# Autodesk Inventor assembly: NDV-1000 Center 01
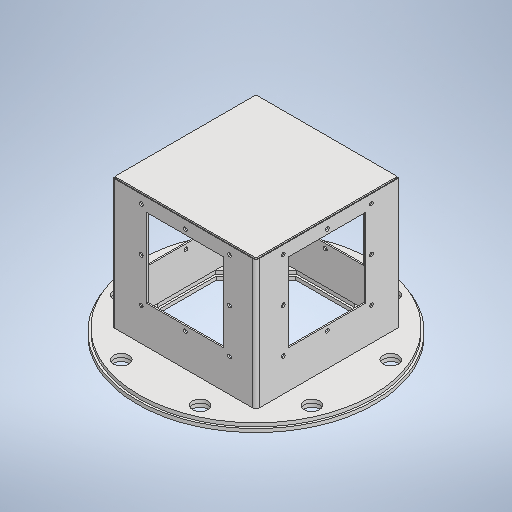
[picture p0: Inventor's stored thumbnail of the model, 512x512]
Saved by Autodesk Inventor 2026.2 (Build 302298000, 298)
## iProperties
Created: 2026-05-12
Part Number: NDV-1000 Center 01
Document SubType Name: Assembly
Designer: admin
Stock Number: Центр
Author: admin
## Documents named in this file (5)
- C:\Users\admin\Documents\Inventor\NDV-DistribSystem\DRS_D1200\NDV-1000 Center 01.iam
- C:\Users\admin\Documents\Inventor\NDV-DistribSystem\DRS_D1200\NDV-1103 Center flange 01.ipt
- C:\Users\admin\Documents\Inventor\NDV-DistribSystem\DRS_D1200\NDV-1101 Center wall 01.ipt
- C:\Users\admin\Documents\Inventor\NDV-DistribSystem\DRS_D1200\NDV-1102 Center cap 01.ipt
- C:\Users\admin\Documents\Inventor\NDV-DistribSystem\DRS_D1200\NDV-1104 Center flange top 01.ipt
## Components (5 placed, 4 different names)
1. NDV-1103 Center flange 01:1 — Mate:6, Flush:3, Flush:4, Flush:5, Flush:6, Mate:9, Mate:10, Flush:7, Flush:8
2. NDV-1101 Center wall 01:1 — Mate:10, Rigid:22, Flush:5, Flush:6, Mate:8
3. NDV-1101 Center wall 01:2 — Rigid:22, Mate:7, Mate:9, Mate:10
4. NDV-1102 Center cap 01:1 — Mate:10, Flush:7, Flush:8
5. NDV-1104 Center flange top 01:1 — Mate:6, Flush:3, Flush:4, Mate:7, Mate:8
## Relationships (13: Mate 6, Flush 6, WeldJoint 1)
- Mate:10: NDV-1101 Center wall 01:1 ↔ NDV-1102 Center cap 01:1
- Rigid:22 [WeldJoint]: NDV-1101 Center wall 01:1 ↔ NDV-1101 Center wall 01:2
- Mate:6: NDV-1103 Center flange 01:1 ↔ NDV-1104 Center flange top 01:1
- Flush:3: NDV-1103 Center flange 01:1 ↔ NDV-1104 Center flange top 01:1
- Flush:4: NDV-1103 Center flange 01:1 ↔ NDV-1104 Center flange top 01:1
- Mate:7: NDV-1101 Center wall 01:2 ↔ NDV-1104 Center flange top 01:1
- Flush:5: NDV-1103 Center flange 01:1 ↔ NDV-1101 Center wall 01:1
- Flush:6 (1 mm): NDV-1103 Center flange 01:1 ↔ NDV-1101 Center wall 01:1
- Mate:8: NDV-1101 Center wall 01:1 ↔ NDV-1104 Center flange top 01:1
- Mate:9: NDV-1103 Center flange 01:1 ↔ NDV-1101 Center wall 01:2
- Mate:10 (1 mm): NDV-1103 Center flange 01:1 ↔ NDV-1101 Center wall 01:2
- Flush:7: NDV-1103 Center flange 01:1 ↔ NDV-1102 Center cap 01:1
- Flush:8: NDV-1103 Center flange 01:1 ↔ NDV-1102 Center cap 01:1
